# Autodesk Inventor assembly: Forearm
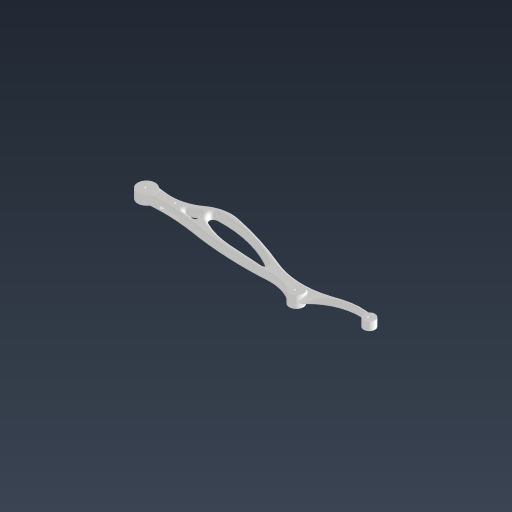
[picture p0: Inventor's stored thumbnail of the model, 512x512]
Saved by Autodesk Inventor 2023 (Build 270158000, 158)
## iProperties
Created: 2023-03-17
Part Number: Forearm
Document SubType Name: Assembly
Designer: valer
Author: valer
## Documents named in this file (3)
- C:\Users\valer\Desktop\str1ker\cad\Forearm.iam
- C:\Users\valer\Desktop\str1ker\cad\Forearm.ipt
- C:\Users\valer\Desktop\str1ker\cad\ForearmBoundingBox.ipt
## Components (2 placed, 2 different names)
1. Forearm:1 — Mate:12, Mate:14, Mate:15, Mate:16, Angle:1
2. ForearmBoundingBox:1 — Mate:17, Angle:1, Angle:2
## Relationships (7: Mate 5, Angle 2)
- Mate:12: Forearm:1
- Mate:14: Forearm:1
- Mate:15: Forearm:1
- Mate:16: Forearm:1
- Mate:17: ForearmBoundingBox:1
- Angle:1 (180 deg): Forearm:1 ↔ ForearmBoundingBox:1
- Angle:2 (0 deg): ForearmBoundingBox:1
